# Autodesk Inventor assembly: for_bool
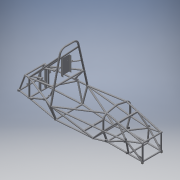
[picture p0: Inventor's stored thumbnail of the model, 180x180]
Saved by Autodesk Inventor 2018.2 (Build 222227000, 227)
## iProperties
Created: 2018-04-27
Part Number: for_bool
Material: 一般
Document SubType Name: Assembly
Designer: ku_sk
Author: ku_sk
## Documents named in this file (4)
- C:\Users\ku_sk\Documents\Inventor\Aero\KS-15\Fr.wing\parts\stay\parts\for_bool.iam
- C:\Users\ku_sk\Documents\Inventor\Aero\KS-15\Fr.wing\parts\stay\parts\frame.ipt
- C:\Users\ku_sk\Documents\Inventor\Aero\KS-15\Fr.wing\parts\stay\parts\bracket1(body).ipt
- C:\Users\ku_sk\Documents\Inventor\Aero\KS-15\Fr.wing\parts\stay\parts\bracket2(body).ipt
## Components (5 placed, 3 different names)
1. frame:1 — メイト:1, メイト:2, メイト:3
2. bracket1(body):1 — 角度:2, 角度:3, フラッシュ:1, フラッシュ:2, フラッシュ:5, フラッシュ:6, フラッシュ:7, フラッシュ:8
3. bracket2(body):1 — 角度:1, フラッシュ:3, フラッシュ:4, フラッシュ:9, フラッシュ:10, フラッシュ:11, フラッシュ:12
4. bracket1(body):2 — フラッシュ:1, フラッシュ:2, フラッシュ:8
5. bracket2(body):2 — フラッシュ:3, フラッシュ:4, フラッシュ:12
## Relationships (18: Flush 12, Mate 3, Angle 3)
- メイト:1 [Mate]: frame:1
- メイト:2 [Mate]: frame:1
- メイト:3 [Mate]: frame:1
- 角度:1 [Angle] (0 deg): bracket2(body):1
- 角度:2 [Angle] (0 deg): bracket1(body):1
- 角度:3 [Angle] (0 deg): bracket1(body):1
- フラッシュ:1 [Flush]: bracket1(body):1 ↔ bracket1(body):2
- フラッシュ:2 [Flush]: bracket1(body):1 ↔ bracket1(body):2
- フラッシュ:3 [Flush]: bracket2(body):1 ↔ bracket2(body):2
- フラッシュ:4 [Flush]: bracket2(body):1 ↔ bracket2(body):2
- フラッシュ:5 [Flush] (1554.866 mm): bracket1(body):1
- フラッシュ:6 [Flush] (-179.5 mm): bracket1(body):1
- フラッシュ:7 [Flush] (-88.003 mm): bracket1(body):1
- フラッシュ:8 [Flush] (359 mm): bracket1(body):1 ↔ bracket1(body):2
- フラッシュ:9 [Flush] (1526.124 mm): bracket2(body):1
- フラッシュ:10 [Flush] (-185.5 mm): bracket2(body):1
- フラッシュ:11 [Flush] (182.171 mm): bracket2(body):1
- フラッシュ:12 [Flush] (371 mm): bracket2(body):1 ↔ bracket2(body):2
